# Autodesk Inventor assembly: 足首_独立ピッチ_1
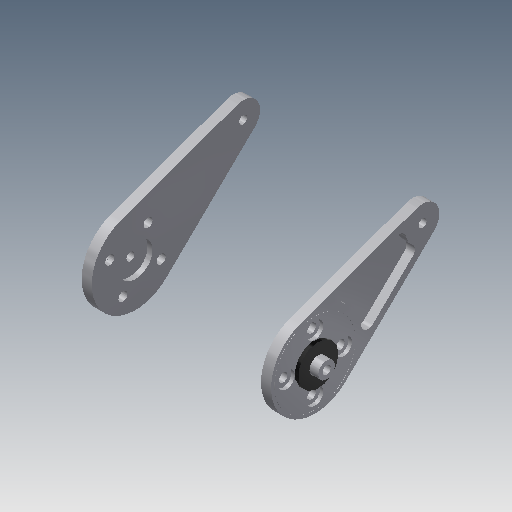
[picture p0: Inventor's stored thumbnail of the model, 512x512]
Saved by Autodesk Inventor 2017.3 (Build 213256000, 256)
## iProperties
Created: 2016-05-04
Part Number: 足首_独立ピッチ_1
Document SubType Name: Assembly
Designer: hiroaki
Mass: 12.0293 g
Surface Area: 78.4578 cm^2
Volume: 4.38559 cm^3
Density: 2.74292 g/cm^3
Author: hiroaki
## Documents named in this file (4)
- C:\Users\haya\Desktop\GankenKun0_5\下半身\足首\足首_独立ピッチ_1.iam
- C:\Users\haya\Desktop\GankenKun0_5\下半身\足首\足首_独立ピッチ_1_1.ipt
- C:\Users\haya\Desktop\GankenKun0_5\下半身\足首\足首_独立ピッチ_1_2.ipt
- C:\Users\haya\Desktop\GankenKun0_5\既製品\CC-0512-10B.ipt
## Components (6 placed, 3 different names)
1. 足首_独立ピッチ_1_1:1 — 挿入:1, 挿入:2, メイト:2, メイト:3, メイト:5, 角度:1
2. 足首_独立ピッチ_1_2:1 — 挿入:1, 挿入:2, メイト:1, メイト:4, 挿入:6
3. 足首_独立ピッチ_1_1:2 — 挿入:3, 挿入:4, メイト:2, メイト:3
4. 足首_独立ピッチ_1_2:2 — 挿入:3, 挿入:4, メイト:1, 挿入:5
5. CC-0512-10B:1 — 挿入:6
6. CC-0512-10B:2 — 挿入:5
## Relationships (12: Insert 6, Mate 5, Angle 1)
- 挿入:1 [Insert]: 足首_独立ピッチ_1_1:1 ↔ 足首_独立ピッチ_1_2:1
- 挿入:2 [Insert]: 足首_独立ピッチ_1_1:1 ↔ 足首_独立ピッチ_1_2:1
- 挿入:3 [Insert]: 足首_独立ピッチ_1_1:2 ↔ 足首_独立ピッチ_1_2:2
- 挿入:4 [Insert]: 足首_独立ピッチ_1_1:2 ↔ 足首_独立ピッチ_1_2:2
- メイト:1 [Mate]: 足首_独立ピッチ_1_2:1 ↔ 足首_独立ピッチ_1_2:2
- メイト:2 [Mate] (50.3 mm): 足首_独立ピッチ_1_1:1 ↔ 足首_独立ピッチ_1_1:2
- メイト:3 [Mate]: 足首_独立ピッチ_1_1:1 ↔ 足首_独立ピッチ_1_1:2
- メイト:4 [Mate]: 足首_独立ピッチ_1_2:1
- メイト:5 [Mate] (25.15 mm): 足首_独立ピッチ_1_1:1
- 角度:1 [Angle] (0 deg): 足首_独立ピッチ_1_1:1
- 挿入:5 [Insert]: 足首_独立ピッチ_1_2:2 ↔ CC-0512-10B:2
- 挿入:6 [Insert]: 足首_独立ピッチ_1_2:1 ↔ CC-0512-10B:1
